# Autodesk Inventor assembly: buoy_mainboard
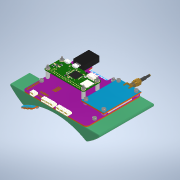
[picture p0: Inventor's stored thumbnail of the model, 180x180]
Saved by Autodesk Inventor 2020.2 (Build 242310000, 310)
## iProperties
Created: 2020-04-10
Part Number: buoy_mainboard
Document SubType Name: Assembly
Designer: agmlego
Mass: 129.366 g
Surface Area: 857.654 cm^2
Volume: 141.767 cm^3
Density: 0.912528 g/cm^3
Author: agmlego
## Documents named in this file (19)
- D:\projects\CreekFleet_AutoBuoy\Mechanical CAD\controls\buoy_mainboard.iam
- D:\projects\CreekFleet_AutoBuoy\Mechanical CAD\controls\buoy_pcb.ipt
- D:\projects\CreekFleet_AutoBuoy\Mechanical CAD\controls\pi-zero\RapberryPiZero.iam
- D:\projects\CreekFleet_AutoBuoy\Mechanical CAD\controls\XT09-SI.ipt
- D:\projects\CreekFleet_AutoBuoy\Mechanical CAD\controls\JST-PH-2\S2B-PH-K-S(LF)(SN)--3DModel-STEP-1.ipt
- D:\projects\CreekFleet_AutoBuoy\Mechanical CAD\controls\ND-105C.ipt
- D:\projects\CreekFleet_AutoBuoy\Mechanical CAD\controls\pololu\dual-g2-hpmd-18v18-24v14-raspberry-pi.ipt
- D:\projects\CreekFleet_AutoBuoy\Mechanical CAD\controls\mainboard_mount.ipt
- D:\projects\CreekFleet_AutoBuoy\Mechanical CAD\hardware\94459A140_BRASS HEAT-SET INSERT FOR PLASTIC.ipt
- D:\projects\CreekFleet_AutoBuoy\Mechanical CAD\controls\rp-sma_end.ipt
- D:\projects\CreekFleet_AutoBuoy\Mechanical CAD\hardware\11mm_standoff.ipt
- \\rackstation\media\documents\Inventor\Content Center Files\R2020\en-US\ANSI B18.3.1M(6)\ANSI B18.3.1M - M2.5x0.45 x 6(1).ipt
- \\rackstation\media\documents\Inventor\Content Center Files\R2020\en-US\ANSI B 18.2.4.1 M(1)\ANSI B 18.2.4.1 M - M2.5 x 0.45Style 1.ipt
- D:\projects\CreekFleet_AutoBuoy\Mechanical CAD\hardware\modem_spacer.ipt
- \\rackstation\media\documents\Inventor\Content Center Files\R2020\en-US\ANSI B18.3.1M(6)\ANSI B18.3.1M - M3x0.5 x 12(1).ipt
- D:\projects\CreekFleet_AutoBuoy\Mechanical CAD\controls\DS3231_RTC.ipt
- D:\projects\CreekFleet_AutoBuoy\Mechanical CAD\hardware\94459A120_BRASS HEAT-SET INSERT FOR PLASTIC.ipt
- \\rackstation\media\documents\Inventor\Content Center Files\R2020\en-US\ANSI B18.3.1M(6)\ANSI B18.3.1M - M2x0.4 x 5(1).ipt
- \\rackstation\media\documents\Inventor\Content Center Files\R2020\en-US\ANSI B18.3.1M(6)\ANSI B18.3.1M - M3x0.5 x 8(1).ipt
## Components (56 placed, 25 different names)
1. modem_spacer:4 — Insert:33
2. modem_spacer:3 — Insert:35, Insert:37
3. modem_spacer:2 — Insert:36, Insert:38
4. modem_spacer:1 — Insert:34
5. 94459A140_BRASS HEAT-SET INSERT FOR PLASTIC:6 — Insert:6
6. 94459A140_BRASS HEAT-SET INSERT FOR PLASTIC:5 — Insert:7
7. 94459A140_BRASS HEAT-SET INSERT FOR PLASTIC:4 — Insert:5
8. 94459A140_BRASS HEAT-SET INSERT FOR PLASTIC:3 — Insert:4
9. XT09-SI:1 — Insert:8, Insert:37, Insert:38, Insert:39, Insert:40, Insert:41, Insert:42
10. rp-sma_end:1 — Insert:8
11. Forged Socket Head Cap Screw - Metric M3x0.5 x 12:1 — Insert:39
12. Forged Socket Head Cap Screw - Metric M3x0.5 x 12:2 — Insert:40
13. Forged Socket Head Cap Screw - Metric M3x0.5 x 12:3 — Insert:41
14. Forged Socket Head Cap Screw - Metric M3x0.5 x 12:4 — Insert:42
15. Forged Socket Head Cap Screw - Metric M3x0.5 x 8:1 — Insert:43
16. Forged Socket Head Cap Screw - Metric M3x0.5 x 8:2 — Insert:44
17. 94459A140_BRASS HEAT-SET INSERT FOR PLASTIC:1
18. 94459A140_BRASS HEAT-SET INSERT FOR PLASTIC:2
19. mainboard_mount:1 — Insert:1, Angle:1, Insert:4, Insert:5, Insert:6, Insert:7, Insert:45, Insert:46
20. buoy_pcb:1 — Mate:1, Flush:1, Flush:2, Mate:8, Mate:9, Mate:10, Mate:11, Mate:12, Mate:13, Mate:14, Mate:15, Tangent:1, Tangent:2, Tangent:3, Tangent:4, Tangent:5, Tangent:6, Tangent:7, Tangent:8, Tangent:9, Tangent:10, Tangent:11, Tangent:12, Insert:1, Angle:1, Insert:9, Insert:10, Insert:11, Insert:12, Insert:19, Insert:20, Insert:21, Insert:22, Insert:23, Insert:24, Insert:31, Insert:32, Insert:33, Insert:34, Insert:35, Insert:36, Insert:43, Insert:44
21. CAN — Mate:15, Tangent:1, Tangent:2, Tangent:3
22. CURR — Mate:8, Flush:8, Tangent:4, Tangent:12
23. FLT — Mate:9, Flush:7, Flush:8, Tangent:11
24. SLP — Mate:10, Flush:6, Flush:7, Tangent:10
25. DIR — Mate:11, Flush:5, Flush:6, Tangent:9
26. PORT LED — Mate:12, Flush:4, Flush:5, Tangent:8
27. STAR LED — Mate:13, Flush:3, Flush:4, Tangent:7
28. ALLROUND LED — Mate:14, Flush:3, Tangent:5, Tangent:6
29. Hex Nut Metric M2.5 x 0.45:1 — Insert:27
30. Hex Nut Metric M2.5 x 0.45:4 — Insert:30
31. Hex Nut Metric M2.5 x 0.45:3 — Insert:29
32. Hex Nut Metric M2.5 x 0.45:2 — Insert:28
33. Forged Socket Head Cap Screw - Metric M2.5x0.45 x 6:5 — Insert:23
34. Forged Socket Head Cap Screw - Metric M2.5x0.45 x 6:6 — Insert:24
35. RapberryPiZero:1 [sub-assembly] — Mate:16, Mate:17, Mate:18, Insert:25, Insert:26, Insert:27, Insert:28, Insert:29, Insert:30
36. ND-105C:1 — Mate:16, Mate:17, Mate:18
37. 11mm_standoff:5 — Insert:20
38. 11mm_standoff:6 — Insert:19
39. 11mm_standoff:7 — Insert:22, Insert:25
40. 11mm_standoff:8 — Insert:21, Insert:26
41. Hex Nut Metric M2.5 x 0.45:5 — Insert:31
42. Hex Nut Metric M2.5 x 0.45:6 — Insert:32
43. dual-g2-hpmd-18v18-24v14-raspberry-pi:1 — Insert:13, Insert:14, Insert:15, Insert:16, Insert:17, Insert:18
44. 11mm_standoff:1 — Insert:12, Insert:13
45. 11mm_standoff:2 — Insert:11
46. 11mm_standoff:3 — Insert:10, Insert:14
47. 11mm_standoff:4 — Insert:9
48. Forged Socket Head Cap Screw - Metric M2.5x0.45 x 6:1 — Insert:15
49. Forged Socket Head Cap Screw - Metric M2.5x0.45 x 6:2 — Insert:16
50. Forged Socket Head Cap Screw - Metric M2.5x0.45 x 6:3 — Insert:17
51. Forged Socket Head Cap Screw - Metric M2.5x0.45 x 6:4 — Insert:18
52. Forged Socket Head Cap Screw - Metric M2x0.4 x 5:1 — Insert:50
53. Forged Socket Head Cap Screw - Metric M2x0.4 x 5:2 — Insert:51
54. DS3231_RTC:1 — Insert:48, Insert:49, Insert:50, Insert:51
55. 94459A120_BRASS HEAT-SET INSERT FOR PLASTIC:2 — Insert:46, Insert:48
56. 94459A120_BRASS HEAT-SET INSERT FOR PLASTIC:3 — Insert:45, Insert:49
## Relationships (81: Insert 48, Mate 12, Tangent 12, Flush 8, Angle 1)
- Mate:1: buoy_pcb:1
- Flush:1: buoy_pcb:1
- Flush:2: buoy_pcb:1
- Mate:8: buoy_pcb:1 ↔ CURR
- Mate:9: buoy_pcb:1 ↔ FLT
- Mate:10: buoy_pcb:1 ↔ SLP
- Mate:11: buoy_pcb:1 ↔ DIR
- Mate:12: buoy_pcb:1 ↔ PORT LED
- Mate:13: buoy_pcb:1 ↔ STAR LED
- Mate:14: buoy_pcb:1 ↔ ALLROUND LED
- Mate:15: buoy_pcb:1 ↔ CAN
- Tangent:1: buoy_pcb:1 ↔ CAN
- Tangent:2: buoy_pcb:1 ↔ CAN
- Tangent:3 (0.6 mm): buoy_pcb:1 ↔ CAN
- Flush:3: STAR LED ↔ ALLROUND LED
- Flush:4: PORT LED ↔ STAR LED
- Flush:5: DIR ↔ PORT LED
- Flush:6: SLP ↔ DIR
- Flush:7: FLT ↔ SLP
- Flush:8: CURR ↔ FLT
- Tangent:4: buoy_pcb:1 ↔ CURR
- Tangent:5: buoy_pcb:1 ↔ ALLROUND LED
- Tangent:6 (0.6 mm): buoy_pcb:1 ↔ ALLROUND LED
- Tangent:7 (0.6 mm): buoy_pcb:1 ↔ STAR LED
- Tangent:8 (0.6 mm): buoy_pcb:1 ↔ PORT LED
- Tangent:9 (0.6 mm): buoy_pcb:1 ↔ DIR
- Tangent:10 (0.6 mm): buoy_pcb:1 ↔ SLP
- Tangent:11 (0.6 mm): buoy_pcb:1 ↔ FLT
- Tangent:12 (0.6 mm): buoy_pcb:1 ↔ CURR
- Mate:16: RapberryPiZero:1 ↔ ND-105C:1
- Mate:17: RapberryPiZero:1 ↔ ND-105C:1
- Mate:18: RapberryPiZero:1 ↔ ND-105C:1
- Insert:1: mainboard_mount:1 ↔ buoy_pcb:1
- Angle:1 (0 deg): mainboard_mount:1 ↔ buoy_pcb:1
- Insert:4: 94459A140_BRASS HEAT-SET INSERT FOR PLASTIC:3 ↔ mainboard_mount:1
- Insert:5: 94459A140_BRASS HEAT-SET INSERT FOR PLASTIC:4 ↔ mainboard_mount:1
- Insert:6: 94459A140_BRASS HEAT-SET INSERT FOR PLASTIC:6 ↔ mainboard_mount:1
- Insert:7: 94459A140_BRASS HEAT-SET INSERT FOR PLASTIC:5 ↔ mainboard_mount:1
- Insert:8: XT09-SI:1 ↔ rp-sma_end:1
- Insert:9: buoy_pcb:1 ↔ 11mm_standoff:4
- Insert:10: buoy_pcb:1 ↔ 11mm_standoff:3
- Insert:11: buoy_pcb:1 ↔ 11mm_standoff:2
- Insert:12: buoy_pcb:1 ↔ 11mm_standoff:1
- Insert:13: dual-g2-hpmd-18v18-24v14-raspberry-pi:1 ↔ 11mm_standoff:1
- Insert:14: dual-g2-hpmd-18v18-24v14-raspberry-pi:1 ↔ 11mm_standoff:3
- Insert:15: dual-g2-hpmd-18v18-24v14-raspberry-pi:1 ↔ Forged Socket Head Cap Screw - Metric M2.5x0.45 x 6:1
- Insert:16: dual-g2-hpmd-18v18-24v14-raspberry-pi:1 ↔ Forged Socket Head Cap Screw - Metric M2.5x0.45 x 6:2
- Insert:17: dual-g2-hpmd-18v18-24v14-raspberry-pi:1 ↔ Forged Socket Head Cap Screw - Metric M2.5x0.45 x 6:3
- Insert:18: dual-g2-hpmd-18v18-24v14-raspberry-pi:1 ↔ Forged Socket Head Cap Screw - Metric M2.5x0.45 x 6:4
- Insert:19: buoy_pcb:1 ↔ 11mm_standoff:6
- Insert:20: buoy_pcb:1 ↔ 11mm_standoff:5
- Insert:21: buoy_pcb:1 ↔ 11mm_standoff:8
- Insert:22: buoy_pcb:1 ↔ 11mm_standoff:7
- Insert:23: buoy_pcb:1 ↔ Forged Socket Head Cap Screw - Metric M2.5x0.45 x 6:5
- Insert:24: buoy_pcb:1 ↔ Forged Socket Head Cap Screw - Metric M2.5x0.45 x 6:6
- Insert:25: RapberryPiZero:1 ↔ 11mm_standoff:7
- Insert:26: RapberryPiZero:1 ↔ 11mm_standoff:8
- Insert:27: Hex Nut Metric M2.5 x 0.45:1 ↔ RapberryPiZero:1
- Insert:28: Hex Nut Metric M2.5 x 0.45:2 ↔ RapberryPiZero:1
- Insert:29: Hex Nut Metric M2.5 x 0.45:3 ↔ RapberryPiZero:1
- Insert:30: Hex Nut Metric M2.5 x 0.45:4 ↔ RapberryPiZero:1
- Insert:31: buoy_pcb:1 ↔ Hex Nut Metric M2.5 x 0.45:5
- Insert:32: buoy_pcb:1 ↔ Hex Nut Metric M2.5 x 0.45:6
- Insert:33: modem_spacer:4 ↔ buoy_pcb:1
- Insert:34: modem_spacer:1 ↔ buoy_pcb:1
- Insert:35: modem_spacer:3 ↔ buoy_pcb:1
- Insert:36: modem_spacer:2 ↔ buoy_pcb:1
- Insert:37: modem_spacer:3 ↔ XT09-SI:1
- Insert:38: modem_spacer:2 ↔ XT09-SI:1
- Insert:39: XT09-SI:1 ↔ Forged Socket Head Cap Screw - Metric M3x0.5 x 12:1
- Insert:40: XT09-SI:1 ↔ Forged Socket Head Cap Screw - Metric M3x0.5 x 12:2
- Insert:41: XT09-SI:1 ↔ Forged Socket Head Cap Screw - Metric M3x0.5 x 12:3
- Insert:42: XT09-SI:1 ↔ Forged Socket Head Cap Screw - Metric M3x0.5 x 12:4
- Insert:43: Forged Socket Head Cap Screw - Metric M3x0.5 x 8:1 ↔ buoy_pcb:1
- Insert:44: Forged Socket Head Cap Screw - Metric M3x0.5 x 8:2 ↔ buoy_pcb:1
- Insert:45: mainboard_mount:1 ↔ 94459A120_BRASS HEAT-SET INSERT FOR PLASTIC:3
- Insert:46: mainboard_mount:1 ↔ 94459A120_BRASS HEAT-SET INSERT FOR PLASTIC:2
- Insert:48: DS3231_RTC:1 ↔ 94459A120_BRASS HEAT-SET INSERT FOR PLASTIC:2
- Insert:49: DS3231_RTC:1 ↔ 94459A120_BRASS HEAT-SET INSERT FOR PLASTIC:3
- Insert:50: Forged Socket Head Cap Screw - Metric M2x0.4 x 5:1 ↔ DS3231_RTC:1
- Insert:51: Forged Socket Head Cap Screw - Metric M2x0.4 x 5:2 ↔ DS3231_RTC:1
